# Autodesk Inventor assembly: New Assembly
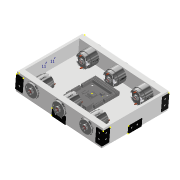
[picture p0: Inventor's stored thumbnail of the model, 180x180]
Saved by Autodesk Inventor 2020 (Build 240168000, 168)
## iProperties
Created: 2020-03-05
Part Number: New Assembly
Document SubType Name: Assembly
Designer: HP
Author: HP
## Documents named in this file (6)
- C:\Users\HP\Desktop\New Assembly.iam
- C:\Users\HP\Desktop\Engineering Exploration\Engineering Exploration Course Project.ipt
- C:\Users\HP\Documents\BME\exploration\arduino.ipt
- C:\Users\HP\Desktop\Engineering Exploration\DC_Motor_1030048_C9000.ipt
- C:\Users\HP\Desktop\Engineering Exploration\L Clamp.ipt
- C:\Users\HP\Desktop\ultrasonic sensor.ipt
## Components (17 placed, 5 different names)
1. Engineering Exploration Course Project:1 — Rigid:1, Rigid:3, Rigid:4, Rigid:5, Rigid:6, Mate:4, Mate:5, Mate:6, Mate:7, Mate:8, Mate:9, Rotational:1, Rotational:2, Rotational:3, Rigid:7, Rotational:4, Rotational:5, Rigid:8, Rigid:9, Rigid:10, Rigid:11, Rigid:12
2. arduino:1 — Rigid:1
3. DC_Motor_1030048_C9000:1 — Mate:5, Rotational:4
4. DC_Motor_1030048_C9000:4 — Mate:6, Rotational:5
5. DC_Motor_1030048_C9000:6 — Mate:4, Rigid:7
6. L Clamp:2 — Rigid:5
7. L Clamp:3 — Rigid:4
8. L Clamp:4 — Rigid:3
9. L Clamp:5 — Rigid:6
10. DC_Motor_1030048_C9000:7 — Mate:7, Rotational:2
11. DC_Motor_1030048_C9000:8 — Mate:9, Rotational:3
12. DC_Motor_1030048_C9000:9 — Mate:8, Rotational:1
13. L Clamp:6 — Rigid:9
14. L Clamp:7 — Rigid:8
15. L Clamp:8 — Rigid:10
16. L Clamp:9 — Rigid:11
17. ultrasonic sensor:1 — Rigid:12
## Relationships (22: WeldJoint 11, Mate 6, RevoluteJoint 5)
- Rigid:1 [WeldJoint]: Engineering Exploration Course Project:1 ↔ arduino:1
- Rigid:3 [WeldJoint]: Engineering Exploration Course Project:1 ↔ L Clamp:4
- Rigid:4 [WeldJoint]: Engineering Exploration Course Project:1 ↔ L Clamp:3
- Rigid:5 [WeldJoint]: Engineering Exploration Course Project:1 ↔ L Clamp:2
- Rigid:6 [WeldJoint]: Engineering Exploration Course Project:1 ↔ L Clamp:5
- Mate:4: Engineering Exploration Course Project:1 ↔ DC_Motor_1030048_C9000:6
- Mate:5: Engineering Exploration Course Project:1 ↔ DC_Motor_1030048_C9000:1
- Mate:6: Engineering Exploration Course Project:1 ↔ DC_Motor_1030048_C9000:4
- Mate:7: Engineering Exploration Course Project:1 ↔ DC_Motor_1030048_C9000:7
- Mate:8: Engineering Exploration Course Project:1 ↔ DC_Motor_1030048_C9000:9
- Mate:9: Engineering Exploration Course Project:1 ↔ DC_Motor_1030048_C9000:8
- Rotational:1 [RevoluteJoint]: Engineering Exploration Course Project:1 ↔ DC_Motor_1030048_C9000:9
- Rotational:2 [RevoluteJoint]: Engineering Exploration Course Project:1 ↔ DC_Motor_1030048_C9000:7
- Rotational:3 [RevoluteJoint]: Engineering Exploration Course Project:1 ↔ DC_Motor_1030048_C9000:8
- Rigid:7 [WeldJoint]: Engineering Exploration Course Project:1 ↔ DC_Motor_1030048_C9000:6
- Rotational:4 [RevoluteJoint]: Engineering Exploration Course Project:1 ↔ DC_Motor_1030048_C9000:1
- Rotational:5 [RevoluteJoint]: Engineering Exploration Course Project:1 ↔ DC_Motor_1030048_C9000:4
- Rigid:8 [WeldJoint]: Engineering Exploration Course Project:1 ↔ L Clamp:7
- Rigid:9 [WeldJoint]: Engineering Exploration Course Project:1 ↔ L Clamp:6
- Rigid:10 [WeldJoint]: Engineering Exploration Course Project:1 ↔ L Clamp:8
- Rigid:11 [WeldJoint]: Engineering Exploration Course Project:1 ↔ L Clamp:9
- Rigid:12 [WeldJoint]: Engineering Exploration Course Project:1 ↔ ultrasonic sensor:1
